# Autodesk Inventor assembly: Mecanum_Assembly
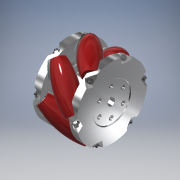
[picture p0: Inventor's stored thumbnail of the model, 180x180]
Saved by Autodesk Inventor 2018 (Build 220112000, 112)
## iProperties
Created: 2017-09-05
Part Number: Mecanum_Assembly
Document SubType Name: Assembly
Designer: P136265
Author: P136265
## Documents named in this file (11)
- C:\Users\P136265\Documents\GitHub\mecanum-cad\Mecanum_Assembly.iam
- C:\Users\P136265\Documents\GitHub\mecanum-cad\roller 8-19-6 bearing.ipt
- C:\Users\P136265\Documents\GitHub\mecanum-cad\MecanumShaft.ipt
- C:\Users\P136265\Documents\GitHub\mecanum-cad\PE_Sleeve.ipt
- C:\Users\P136265\Documents\GitHub\mecanum-cad\CheekPlate.ipt
- C:\Users\P136265\Documents\GitHub\mecanum-cad\MecanumHub.ipt
- C:\Users\P136265\Documents\GitHub\mecanum-cad\Washer.ipt
- C:\Users\P136265\Documents\Inventor\Content Center Files\R2018\en-US\AS 1474(1)\AS 1474 - M8(1).ipt
- C:\Users\P136265\Documents\Inventor\Content Center Files\R2018\en-US\AS 1420\AS 1420 - 1973 - M6 x 30.ipt
- C:\Users\P136265\Documents\Inventor\Content Center Files\R2018\en-US\AS 1112 (2)\AS 1112 - M6  Type 5.ipt
- C:\Users\P136265\Documents\Inventor\Content Center Files\R2018\en-US\DIN 625 SKF(5)\DIN 625 SKF - SKF 619_8-2RS1.ipt
## Components (105 placed, 10 different names)
1. CheekPlate:2 — Mate:14, Mate:15, Mate:23, Mate:28, Mate:29, Mate:41, Mate:42
2. MecanumHub:1 — Mate:27, Mate:31, Mate:40, Mate:41, Mate:42, Mate:43
3. CheekPlate:3 — Mate:40, Mate:43
4. roller 8-19-6 bearing:1 — Mate:1, Angle:1, Mate:2, Mate:3, Mate:4, Insert:1, Insert:2, Angle:2, Mate:9, Mate:15, Mate:32, Mate:34
5. MecanumShaft:1 — Angle:2, Mate:9, Mate:10, Mate:20, Mate:22, Mate:36, Mate:38
6. PE_Sleeve:1 — Mate:3, Mate:4
7. Washer:1 — Mate:5, Mate:6, Mate:33
8. Washer:2 — Mate:7, Mate:8, Mate:10, Mate:35
9. DIN 625 SKF- with two RS1 seals SKF 619/8-2RS1:1 — Insert:1, Mate:7, Mate:8
10. DIN 625 SKF- with two RS1 seals SKF 619/8-2RS1:2 — Insert:2, Mate:5, Mate:6
11. DIN 625 SKF- with two RS1 seals SKF 619/8-2RS1:13 — Mate:32, Mate:33, Mate:37
12. DIN 625 SKF- with two RS1 seals SKF 619/8-2RS1:19 — Mate:34, Mate:35, Mate:39
13. Washer:13 — Mate:36, Mate:37
14. Washer:14 — Mate:38, Mate:39
15. roller 8-19-6 bearing:2
16. MecanumShaft:2
17. PE_Sleeve:2
18. Washer:3
19. Washer:4
20. DIN 625 SKF- with two RS1 seals SKF 619/8-2RS1:3
21. DIN 625 SKF- with two RS1 seals SKF 619/8-2RS1:4
22. DIN 625 SKF- with two RS1 seals SKF 619/8-2RS1:14
23. DIN 625 SKF- with two RS1 seals SKF 619/8-2RS1:20
24. Washer:15
25. Washer:20
26. roller 8-19-6 bearing:3
27. MecanumShaft:3
28. PE_Sleeve:3
29. Washer:5
30. Washer:6
31. DIN 625 SKF- with two RS1 seals SKF 619/8-2RS1:5
32. DIN 625 SKF- with two RS1 seals SKF 619/8-2RS1:6
33. DIN 625 SKF- with two RS1 seals SKF 619/8-2RS1:15
34. DIN 625 SKF- with two RS1 seals SKF 619/8-2RS1:21
35. Washer:16
36. Washer:21
37. roller 8-19-6 bearing:4
38. MecanumShaft:4 — Mate:14
39. PE_Sleeve:4
40. Washer:7
41. Washer:8
42. DIN 625 SKF- with two RS1 seals SKF 619/8-2RS1:7
43. DIN 625 SKF- with two RS1 seals SKF 619/8-2RS1:8
44. DIN 625 SKF- with two RS1 seals SKF 619/8-2RS1:16
45. DIN 625 SKF- with two RS1 seals SKF 619/8-2RS1:22
46. Washer:17
47. Washer:22
48. roller 8-19-6 bearing:5
49. MecanumShaft:5
50. PE_Sleeve:5
51. Washer:9
52. Washer:10
53. DIN 625 SKF- with two RS1 seals SKF 619/8-2RS1:9
54. DIN 625 SKF- with two RS1 seals SKF 619/8-2RS1:10
55. DIN 625 SKF- with two RS1 seals SKF 619/8-2RS1:17
56. DIN 625 SKF- with two RS1 seals SKF 619/8-2RS1:23
57. Washer:18
58. Washer:23
59. roller 8-19-6 bearing:6
60. MecanumShaft:6
61. PE_Sleeve:6
62. Washer:11
63. Washer:12
64. DIN 625 SKF- with two RS1 seals SKF 619/8-2RS1:11
65. DIN 625 SKF- with two RS1 seals SKF 619/8-2RS1:12
66. DIN 625 SKF- with two RS1 seals SKF 619/8-2RS1:18
67. DIN 625 SKF- with two RS1 seals SKF 619/8-2RS1:24
68. Washer:19
69. Washer:24
70. AS 1474 - Metric M8:13 — Mate:20
71. AS 1474 - Metric M8:19 — Mate:22, Mate:23
72. AS 1474 - Metric M8:14
73. AS 1474 - Metric M8:20
74. AS 1474 - Metric M8:15
75. AS 1474 - Metric M8:21
76. AS 1474 - Metric M8:16
77. AS 1474 - Metric M8:22
78. AS 1474 - Metric M8:17
79. AS 1474 - Metric M8:23
80. AS 1474 - Metric M8:18
81. AS 1474 - Metric M8:24
82. AS 1420 - Metric M6 x 30:13 — Mate:26
83. AS 1420 - Metric M6 x 30:14
84. AS 1420 - Metric M6 x 30:15
85. AS 1420 - Metric M6 x 30:16
86. AS 1420 - Metric M6 x 30:17
87. AS 1420 - Metric M6 x 30:18
88. AS 1112 (2) - Metric M6  Type 5:13 — Mate:26, Mate:27
89. AS 1112 (2) - Metric M6  Type 5:14
90. AS 1112 (2) - Metric M6  Type 5:15
91. AS 1112 (2) - Metric M6  Type 5:16
92. AS 1112 (2) - Metric M6  Type 5:17
93. AS 1112 (2) - Metric M6  Type 5:18
94. AS 1420 - Metric M6 x 30:19 — Mate:28, Mate:29, Mate:30
95. AS 1420 - Metric M6 x 30:20
96. AS 1420 - Metric M6 x 30:21
97. AS 1420 - Metric M6 x 30:22
98. AS 1420 - Metric M6 x 30:23
99. AS 1420 - Metric M6 x 30:24
100. AS 1112 (2) - Metric M6  Type 5:19 — Mate:30, Mate:31
101. AS 1112 (2) - Metric M6  Type 5:20
102. AS 1112 (2) - Metric M6  Type 5:21
103. AS 1112 (2) - Metric M6  Type 5:22
104. AS 1112 (2) - Metric M6  Type 5:23
105. AS 1112 (2) - Metric M6  Type 5:24
## Component patterns: (6 elements, first: roller 8-19-6 bearing:1 + MecanumShaft:1 + PE_Sleeve:1 + Washer:1 + Washer:2 + DIN 625 SKF- with two RS1 seals SKF 619/8-2RS1:1 + DIN 625 SKF- with two RS1 seals SKF 619/8-2RS1:2 + DIN 625 SKF- with two RS1 seals SKF 619/8-2RS1:13 + DIN 625 SKF- with two RS1 seals SKF 619/8-2RS1:19 + Washer:13 + Washer:14), (6 elements, first: AS 1474 - Metric M8:13 + AS 1474 - Metric M8:19), (6 elements, first: AS 1420 - Metric M6 x 30:13), (6 elements, first: AS 1112 (2) - Metric M6  Type 5:13), (6 elements, first: AS 1420 - Metric M6 x 30:19), (6 elements, first: AS 1112 (2) - Metric M6  Type 5:19)
## Relationships (37: Mate 33, Angle 2, Insert 2)
- Mate:1 (75 mm): roller 8-19-6 bearing:1
- Angle:1 (45 deg): roller 8-19-6 bearing:1
- Mate:2: roller 8-19-6 bearing:1
- Mate:3: roller 8-19-6 bearing:1 ↔ PE_Sleeve:1
- Mate:4: roller 8-19-6 bearing:1 ↔ PE_Sleeve:1
- Insert:1: roller 8-19-6 bearing:1 ↔ DIN 625 SKF- with two RS1 seals SKF 619/8-2RS1:1
- Insert:2: roller 8-19-6 bearing:1 ↔ DIN 625 SKF- with two RS1 seals SKF 619/8-2RS1:2
- Mate:5: Washer:1 ↔ DIN 625 SKF- with two RS1 seals SKF 619/8-2RS1:2
- Mate:6: Washer:1 ↔ DIN 625 SKF- with two RS1 seals SKF 619/8-2RS1:2
- Mate:7: Washer:2 ↔ DIN 625 SKF- with two RS1 seals SKF 619/8-2RS1:1
- Mate:8: Washer:2 ↔ DIN 625 SKF- with two RS1 seals SKF 619/8-2RS1:1
- Angle:2 (0 deg): roller 8-19-6 bearing:1 ↔ MecanumShaft:1
- Mate:9: roller 8-19-6 bearing:1 ↔ MecanumShaft:1
- Mate:10 (25 mm): MecanumShaft:1 ↔ Washer:2
- Mate:14: CheekPlate:2 ↔ MecanumShaft:4
- Mate:15: CheekPlate:2 ↔ roller 8-19-6 bearing:1
- Mate:20: MecanumShaft:1 ↔ AS 1474 - Metric M8:13
- Mate:22: MecanumShaft:1 ↔ AS 1474 - Metric M8:19
- Mate:23: CheekPlate:2 ↔ AS 1474 - Metric M8:19
- Mate:26: AS 1420 - Metric M6 x 30:13 ↔ AS 1112 (2) - Metric M6  Type 5:13
- Mate:27: MecanumHub:1 ↔ AS 1112 (2) - Metric M6  Type 5:13
- Mate:28: CheekPlate:2 ↔ AS 1420 - Metric M6 x 30:19
- Mate:29: CheekPlate:2 ↔ AS 1420 - Metric M6 x 30:19
- Mate:30: AS 1420 - Metric M6 x 30:19 ↔ AS 1112 (2) - Metric M6  Type 5:19
- Mate:31: MecanumHub:1 ↔ AS 1112 (2) - Metric M6  Type 5:19
- Mate:32: roller 8-19-6 bearing:1 ↔ DIN 625 SKF- with two RS1 seals SKF 619/8-2RS1:13
- Mate:33: Washer:1 ↔ DIN 625 SKF- with two RS1 seals SKF 619/8-2RS1:13
- Mate:34: roller 8-19-6 bearing:1 ↔ DIN 625 SKF- with two RS1 seals SKF 619/8-2RS1:19
- Mate:35: Washer:2 ↔ DIN 625 SKF- with two RS1 seals SKF 619/8-2RS1:19
- Mate:36: MecanumShaft:1 ↔ Washer:13
- Mate:37: DIN 625 SKF- with two RS1 seals SKF 619/8-2RS1:13 ↔ Washer:13
- Mate:38: MecanumShaft:1 ↔ Washer:14
- Mate:39: DIN 625 SKF- with two RS1 seals SKF 619/8-2RS1:19 ↔ Washer:14
- Mate:40: MecanumHub:1 ↔ CheekPlate:3
- Mate:41: CheekPlate:2 ↔ MecanumHub:1
- Mate:42: CheekPlate:2 ↔ MecanumHub:1
- Mate:43: MecanumHub:1 ↔ CheekPlate:3
